# Autodesk Inventor assembly: Solar Panel
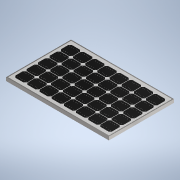
[picture p0: Inventor's stored thumbnail of the model, 180x180]
Saved by Autodesk Inventor 2020 (Build 240168000, 168)
## iProperties
Created: 2020-06-26
Part Number: Solar Panel
Document SubType Name: Assembly
Designer: Abbas
Author: Abbas
## Documents named in this file (4)
- C:\Users\LENOVO\Desktop\Graduation Project\Fish Farming Unit\solar panel\Solar Panel.iam
- C:\Users\LENOVO\Desktop\Graduation Project\Fish Farming Unit\solar panel\frame.ipt
- C:\Users\LENOVO\Desktop\Graduation Project\Fish Farming Unit\solar panel\panel.ipt
- C:\Users\LENOVO\Desktop\Graduation Project\Fish Farming Unit\solar panel\panel2.ipt
## Components (3 placed, 3 different names)
1. frame:2 — Mate:1, Mate:2
2. panel:1 — Mate:1, Mate:2, Mate:3
3. panel2:1 — Mate:3
## Relationships (3: Mate 3)
- Mate:1: frame:2 ↔ panel:1
- Mate:2: frame:2 ↔ panel:1
- Mate:3: panel:1 ↔ panel2:1
